# Autodesk Inventor assembly: Pakiet_zagrzany
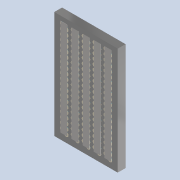
[picture p0: Inventor's stored thumbnail of the model, 180x180]
Saved by Autodesk Inventor 2021.3 (Build 253353000, 353)
## iProperties
Created: 2023-05-23
Part Number: Pakiet_zagrzany
Document SubType Name: Assembly
Designer: User
Author: User
## Documents named in this file (7)
- E:\Inventor\Projekty\Modele Robotyzacja Procesów\Pakiet_zagrzany.iam
- E:\Inventor\Projekty\Modele Robotyzacja Procesów\Model_Sita.ipt
- E:\Inventor\Projekty\Modele Robotyzacja Procesów\Model_Ogniwa.ipt
- E:\Inventor\Projekty\Modele Robotyzacja Procesów\tasiemka_do_zgrzewania_1.ipt
- tasiemka_do_zgrzewania_1.ipt
- E:\Inventor\Projekty\Modele Robotyzacja Procesów\tasiemka_do_zgrzewania_2.ipt
- E:\Inventor\Projekty\Modele Robotyzacja Procesów\tasiemka_do_zgrzewania_3.ipt
## Components (212 placed, 5 different names)
1. Model_Sita:1 — Zestawiające:1, Równoległe:1, Zestawiające:2, Równoległe:2, Równoległe:3, Równoległe:4, Równoległe:5, Równoległe:6, Zestawiające:13, Zestawiające:14, Zestawiające:15, Zestawiające:16, Zestawiające:17, Równoległe:11, Równoległe:16, Równoległe:17
2. tasiemka_do_zgrzewania_1:1 — Zestawiające:4, Równoległe:4, Równoległe:6, Równoległe:8, Równoległe:9, Zestawiające:8
3. tasiemka_do_zgrzewania_1:2 — Zestawiające:3, Równoległe:3, Równoległe:5, Równoległe:7, Równoległe:10, Zestawiające:5
4. tasiemka_do_zgrzewania_2:1 — Zestawiające:14, Równoległe:12, Równoległe:13, Zestawiające:18, Zestawiające:19
5. tasiemka_do_zgrzewania_2:2 — Zestawiające:15, Równoległe:13, Równoległe:14, Zestawiające:19, Zestawiające:20
6. tasiemka_do_zgrzewania_2:3 — Zestawiające:16, Równoległe:14, Równoległe:15, Zestawiające:20
7. tasiemka_do_zgrzewania_2:4 — Zestawiające:17, Równoległe:15, Równoległe:17
8. tasiemka_do_zgrzewania_2:5 — Zestawiające:13, Równoległe:11, Równoległe:12, Równoległe:16, Zestawiające:18
9. tasiemka_do_zgrzewania_3:1 — Równoległe:7, Zestawiające:5, Zestawiające:6, Zestawiające:12
10. tasiemka_do_zgrzewania_3:2 — Równoległe:10, Zestawiające:6, Zestawiające:7, Zestawiające:11
11. tasiemka_do_zgrzewania_3:3 — Równoległe:9, Zestawiające:7, Zestawiające:10
12. tasiemka_do_zgrzewania_3:4 — Równoległe:8, Zestawiające:8, Zestawiające:9
13. Model_Ogniwa:1 — Zestawiające:1, Równoległe:1
14. Model_Ogniwa:2
15. Model_Ogniwa:3
16. Model_Ogniwa:4
17. Model_Ogniwa:5
18. Model_Ogniwa:6
19. Model_Ogniwa:7
20. Model_Ogniwa:8
21. Model_Ogniwa:9
22. Model_Ogniwa:10
23. Model_Ogniwa:11
24. Model_Ogniwa:12
25. Model_Ogniwa:13
26. Model_Ogniwa:14
27. Model_Ogniwa:15
28. Model_Ogniwa:16
29. Model_Ogniwa:17
30. Model_Ogniwa:18
31. Model_Ogniwa:19
32. Model_Ogniwa:20 — Zestawiające:4
33. Model_Ogniwa:21
34. Model_Ogniwa:22
35. Model_Ogniwa:23
36. Model_Ogniwa:24
37. Model_Ogniwa:25
38. Model_Ogniwa:26
39. Model_Ogniwa:27
40. Model_Ogniwa:28
41. Model_Ogniwa:29
42. Model_Ogniwa:30
43. Model_Ogniwa:31
44. Model_Ogniwa:32
45. Model_Ogniwa:33
46. Model_Ogniwa:34
47. Model_Ogniwa:35
48. Model_Ogniwa:36
49. Model_Ogniwa:37
50. Model_Ogniwa:38
51. Model_Ogniwa:39
52. Model_Ogniwa:40
53. Model_Ogniwa:41
54. Model_Ogniwa:42
55. Model_Ogniwa:43
56. Model_Ogniwa:44
57. Model_Ogniwa:45
58. Model_Ogniwa:46
59. Model_Ogniwa:47
60. Model_Ogniwa:48
61. Model_Ogniwa:49
62. Model_Ogniwa:50
63. Model_Ogniwa:51
64. Model_Ogniwa:52
65. Model_Ogniwa:53
66. Model_Ogniwa:54
67. Model_Ogniwa:55
68. Model_Ogniwa:56
69. Model_Ogniwa:57
70. Model_Ogniwa:58
71. Model_Ogniwa:59
72. Model_Ogniwa:60
73. Model_Ogniwa:61
74. Model_Ogniwa:62
75. Model_Ogniwa:63
76. Model_Ogniwa:64
77. Model_Ogniwa:65
78. Model_Ogniwa:66
79. Model_Ogniwa:67
80. Model_Ogniwa:68
81. Model_Ogniwa:69
82. Model_Ogniwa:70
83. Model_Ogniwa:71
84. Model_Ogniwa:72
85. Model_Ogniwa:73
86. Model_Ogniwa:74
87. Model_Ogniwa:75
88. Model_Ogniwa:76
89. Model_Ogniwa:77
90. Model_Ogniwa:78
91. Model_Ogniwa:79 — Zestawiające:11
92. Model_Ogniwa:80
93. Model_Ogniwa:81
94. Model_Ogniwa:82
95. Model_Ogniwa:83
96. Model_Ogniwa:84
97. Model_Ogniwa:85
98. Model_Ogniwa:86
99. Model_Ogniwa:87
100. Model_Ogniwa:88
101. Model_Ogniwa:89
102. Model_Ogniwa:90
103. Model_Ogniwa:91
104. Model_Ogniwa:92
105. Model_Ogniwa:93
106. Model_Ogniwa:94
107. Model_Ogniwa:95
108. Model_Ogniwa:96
109. Model_Ogniwa:97
110. Model_Ogniwa:98
111. Model_Ogniwa:99 — Zestawiające:12
112. Model_Ogniwa:100
113. Model_Ogniwa:101 — Zestawiające:2, Równoległe:2
114. Model_Ogniwa:102
115. Model_Ogniwa:103
116. Model_Ogniwa:104
117. Model_Ogniwa:105
118. Model_Ogniwa:106
119. Model_Ogniwa:107
120. Model_Ogniwa:108
121. Model_Ogniwa:109
122. Model_Ogniwa:110
123. Model_Ogniwa:111
124. Model_Ogniwa:112
125. Model_Ogniwa:113
126. Model_Ogniwa:114
127. Model_Ogniwa:115
128. Model_Ogniwa:116
129. Model_Ogniwa:117
130. Model_Ogniwa:118
131. Model_Ogniwa:119
132. Model_Ogniwa:120 — Zestawiające:9
133. Model_Ogniwa:121
134. Model_Ogniwa:122
135. Model_Ogniwa:123
136. Model_Ogniwa:124
137. Model_Ogniwa:125
138. Model_Ogniwa:126
139. Model_Ogniwa:127
140. Model_Ogniwa:128
141. Model_Ogniwa:129
142. Model_Ogniwa:130
143. Model_Ogniwa:131
144. Model_Ogniwa:132
145. Model_Ogniwa:133
146. Model_Ogniwa:134
147. Model_Ogniwa:135
148. Model_Ogniwa:136
149. Model_Ogniwa:137
150. Model_Ogniwa:138
151. Model_Ogniwa:139 — Zestawiające:10
152. Model_Ogniwa:140
153. Model_Ogniwa:141
154. Model_Ogniwa:142
155. Model_Ogniwa:143
156. Model_Ogniwa:144
157. Model_Ogniwa:145
158. Model_Ogniwa:146
159. Model_Ogniwa:147
160. Model_Ogniwa:148
161. Model_Ogniwa:149
162. Model_Ogniwa:150
163. Model_Ogniwa:151
164. Model_Ogniwa:152
165. Model_Ogniwa:153
166. Model_Ogniwa:154
167. Model_Ogniwa:155
168. Model_Ogniwa:156
169. Model_Ogniwa:157
170. Model_Ogniwa:158
171. Model_Ogniwa:159
172. Model_Ogniwa:160
173. Model_Ogniwa:161
174. Model_Ogniwa:162
175. Model_Ogniwa:163
176. Model_Ogniwa:164
177. Model_Ogniwa:165
178. Model_Ogniwa:166
179. Model_Ogniwa:167
180. Model_Ogniwa:168
181. Model_Ogniwa:169
182. Model_Ogniwa:170
183. Model_Ogniwa:171
184. Model_Ogniwa:172
185. Model_Ogniwa:173
186. Model_Ogniwa:174
187. Model_Ogniwa:175
188. Model_Ogniwa:176
189. Model_Ogniwa:177
190. Model_Ogniwa:178
191. Model_Ogniwa:179
192. Model_Ogniwa:180
193. Model_Ogniwa:181
194. Model_Ogniwa:182
195. Model_Ogniwa:183
196. Model_Ogniwa:184
197. Model_Ogniwa:185
198. Model_Ogniwa:186
199. Model_Ogniwa:187
200. Model_Ogniwa:188
201. Model_Ogniwa:189
202. Model_Ogniwa:190
203. Model_Ogniwa:191
204. Model_Ogniwa:192
205. Model_Ogniwa:193
206. Model_Ogniwa:194
207. Model_Ogniwa:195
208. Model_Ogniwa:196
209. Model_Ogniwa:197
210. Model_Ogniwa:198
211. Model_Ogniwa:199
212. Model_Ogniwa:200 — Zestawiające:3
## Component patterns: (5 elements), (5 elements), (20 elements, first: Model_Ogniwa:1), Szyk komponentów 1:2 (20 elements), Szyk komponentów 1:3 (20 elements), Szyk komponentów 1:4 (20 elements), Szyk komponentów 1:5 (20 elements), (20 elements, first: Model_Ogniwa:101), Szyk komponentów 3:2 (20 elements), Szyk komponentów 3:3 (20 elements), Szyk komponentów 3:4 (20 elements), Szyk komponentów 3:5 (20 elements)
## Relationships (37: Mate 20, Flush 17)
- Zestawiające:1 [Mate]: Model_Sita:1 ↔ Model_Ogniwa:1
- Równoległe:1 [Flush]: Model_Sita:1 ↔ Model_Ogniwa:1
- Zestawiające:2 [Mate]: Model_Sita:1 ↔ Model_Ogniwa:101
- Równoległe:2 [Flush]: Model_Sita:1 ↔ Model_Ogniwa:101
- Zestawiające:3 [Mate]: tasiemka_do_zgrzewania_1:2 ↔ Model_Ogniwa:200
- Równoległe:3 [Flush] (54 mm): Model_Sita:1 ↔ tasiemka_do_zgrzewania_1:2
- Zestawiające:4 [Mate]: tasiemka_do_zgrzewania_1:1 ↔ Model_Ogniwa:20
- Równoległe:4 [Flush] (54 mm): Model_Sita:1 ↔ tasiemka_do_zgrzewania_1:1
- Równoległe:5 [Flush] (60 mm): Model_Sita:1 ↔ tasiemka_do_zgrzewania_1:2
- Równoległe:6 [Flush] (50 mm): Model_Sita:1 ↔ tasiemka_do_zgrzewania_1:1
- Równoległe:7 [Flush]: tasiemka_do_zgrzewania_1:2 ↔ tasiemka_do_zgrzewania_3:1
- Równoległe:8 [Flush]: tasiemka_do_zgrzewania_1:1 ↔ tasiemka_do_zgrzewania_3:4
- Równoległe:9 [Flush]: tasiemka_do_zgrzewania_1:1 ↔ tasiemka_do_zgrzewania_3:3
- Równoległe:10 [Flush]: tasiemka_do_zgrzewania_1:2 ↔ tasiemka_do_zgrzewania_3:2
- Zestawiające:5 [Mate] (10 mm): tasiemka_do_zgrzewania_1:2 ↔ tasiemka_do_zgrzewania_3:1
- Zestawiające:6 [Mate] (15 mm): tasiemka_do_zgrzewania_3:1 ↔ tasiemka_do_zgrzewania_3:2
- Zestawiające:7 [Mate] (20 mm): tasiemka_do_zgrzewania_3:2 ↔ tasiemka_do_zgrzewania_3:3
- Zestawiające:8 [Mate] (10 mm): tasiemka_do_zgrzewania_1:1 ↔ tasiemka_do_zgrzewania_3:4
- Zestawiające:9 [Mate]: tasiemka_do_zgrzewania_3:4 ↔ Model_Ogniwa:120
- Zestawiające:10 [Mate]: tasiemka_do_zgrzewania_3:3 ↔ Model_Ogniwa:139
- Zestawiające:11 [Mate]: tasiemka_do_zgrzewania_3:2 ↔ Model_Ogniwa:79
- Zestawiające:12 [Mate]: tasiemka_do_zgrzewania_3:1 ↔ Model_Ogniwa:99
- Zestawiające:13 [Mate]: Model_Sita:1 ↔ tasiemka_do_zgrzewania_2:5
- Zestawiające:14 [Mate]: Model_Sita:1 ↔ tasiemka_do_zgrzewania_2:1
- Zestawiające:15 [Mate]: Model_Sita:1 ↔ tasiemka_do_zgrzewania_2:2
- Zestawiające:16 [Mate]: Model_Sita:1 ↔ tasiemka_do_zgrzewania_2:3
- Zestawiające:17 [Mate]: Model_Sita:1 ↔ tasiemka_do_zgrzewania_2:4
- Równoległe:11 [Flush] (45 mm): Model_Sita:1 ↔ tasiemka_do_zgrzewania_2:5
- Równoległe:12 [Flush]: tasiemka_do_zgrzewania_2:1 ↔ tasiemka_do_zgrzewania_2:5
- Równoległe:13 [Flush]: tasiemka_do_zgrzewania_2:1 ↔ tasiemka_do_zgrzewania_2:2
- Równoległe:14 [Flush]: tasiemka_do_zgrzewania_2:2 ↔ tasiemka_do_zgrzewania_2:3
- Równoległe:15 [Flush]: tasiemka_do_zgrzewania_2:3 ↔ tasiemka_do_zgrzewania_2:4
- Równoległe:16 [Flush] (65 mm): Model_Sita:1 ↔ tasiemka_do_zgrzewania_2:5
- Równoległe:17 [Flush] (65 mm): Model_Sita:1 ↔ tasiemka_do_zgrzewania_2:4
- Zestawiające:18 [Mate] (44 mm): tasiemka_do_zgrzewania_2:1 ↔ tasiemka_do_zgrzewania_2:5
- Zestawiające:19 [Mate] (44 mm): tasiemka_do_zgrzewania_2:1 ↔ tasiemka_do_zgrzewania_2:2
- Zestawiające:20 [Mate] (44 mm): tasiemka_do_zgrzewania_2:2 ↔ tasiemka_do_zgrzewania_2:3
